# Autodesk Inventor assembly: carro_linear
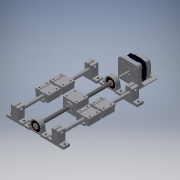
[picture p0: Inventor's stored thumbnail of the model, 180x180]
Saved by Autodesk Inventor 2018 (Build 220112000, 112)
## iProperties
Created: 2018-09-21
Part Number: carro_linear
Material: Genérico
Document SubType Name: Assembly
Designer: Georgines
Author: Georgines
## Documents named in this file (10)
- C:\Users\Georgines\Documents\EstacaoBGA\Peças 3D\carro_linear.iam
- C:\Users\Georgines\Documents\EstacaoBGA\Peças 3D\CastanhaTR8.ipt
- C:\Users\Georgines\Documents\EstacaoBGA\Peças 3D\FusoTrapezoidal_8mmx200mm.ipt
- C:\Users\Georgines\Documents\EstacaoBGA\Peças 3D\kp08.ipt
- C:\Users\Georgines\Documents\EstacaoBGA\Peças 3D\NEMA-17_17HS4401.ipt
- C:\Users\Georgines\Documents\EstacaoBGA\Peças 3D\SCS8UU.iam
- C:\Users\Georgines\Documents\EstacaoBGA\Peças 3D\Sk8.ipt
- C:\Users\Georgines\Documents\EstacaoBGA\Peças 3D\SuporteCastanhaTr8.ipt
- C:\Users\Georgines\Documents\EstacaoBGA\Peças 3D\SuporteLMotorNema17.ipt
- C:\Users\Georgines\Documents\EstacaoBGA\Peças 3D\GuiaLinear_8mmx200mm.ipt
## Components (17 placed, 9 different names)
1. FusoTrapezoidal_8mmx200mm:1 — Coincidência:9, Coincidência:10, Alinhamento:10, Inserir:1
2. kp08:1 — Alinhamento:7, Coincidência:9, Alinhamento:9, Alinhamento:10, Alinhamento:20, Alinhamento:23, Coincidência:13, Coincidência:14
3. kp08:2 — Alinhamento:8, Coincidência:10, Alinhamento:11, Alinhamento:16, Alinhamento:21, Alinhamento:22
4. NEMA-17_17HS4401:1 — Coincidência:11, Coincidência:12
5. GuiaLinear_8mmx200mm:1 — Coincidência:2, Alinhamento:2, Coincidência:4, Alinhamento:4, Coincidência:5, Coincidência:8
6. GuiaLinear_8mmx200mm:2 — Coincidência:1, Alinhamento:1, Coincidência:3, Alinhamento:3, Coincidência:6, Coincidência:7
7. Sk8:1 — Coincidência:1, Alinhamento:1, Alinhamento:7, Alinhamento:9, Alinhamento:23, Coincidência:14
8. Sk8:2 — Coincidência:2, Alinhamento:2, Alinhamento:20, Coincidência:13
9. Sk8:3 — Coincidência:3, Alinhamento:3, Alinhamento:5, Alinhamento:6, Alinhamento:8, Alinhamento:11, Alinhamento:22
10. Sk8:4 — Coincidência:4, Alinhamento:4, Alinhamento:5, Alinhamento:6, Alinhamento:21
11. SCS8UU:1 [sub-assembly] — Coincidência:8, Alinhamento:12, Alinhamento:13, Alinhamento:17, Alinhamento:24
12. SCS8UU:2 [sub-assembly] — Coincidência:7, Alinhamento:14, Alinhamento:15, Alinhamento:17, Alinhamento:24, Coincidência:15
13. SCS8UU:3 [sub-assembly] — Coincidência:5, Alinhamento:12, Alinhamento:13, Alinhamento:18, Alinhamento:19, Alinhamento:25
14. SCS8UU:4 [sub-assembly] — Coincidência:6, Alinhamento:14, Alinhamento:15, Alinhamento:18, Alinhamento:19, Coincidência:15
15. SuporteLMotorNema17:1 — Coincidência:11, Coincidência:12, Alinhamento:16
16. SuporteCastanhaTr8:1 — Coincidência:16, Coincidência:17, Alinhamento:25
17. CastanhaTR8:1 — Inserir:1, Coincidência:16, Coincidência:17
## Relationships (43: Flush 25, Mate 17, Insert 1)
- Coincidência:1 [Mate]: GuiaLinear_8mmx200mm:2 ↔ Sk8:1
- Coincidência:2 [Mate]: GuiaLinear_8mmx200mm:1 ↔ Sk8:2
- Alinhamento:1 [Flush]: GuiaLinear_8mmx200mm:2 ↔ Sk8:1
- Alinhamento:2 [Flush]: GuiaLinear_8mmx200mm:1 ↔ Sk8:2
- Coincidência:3 [Mate]: GuiaLinear_8mmx200mm:2 ↔ Sk8:3
- Coincidência:4 [Mate]: GuiaLinear_8mmx200mm:1 ↔ Sk8:4
- Alinhamento:3 [Flush]: GuiaLinear_8mmx200mm:2 ↔ Sk8:3
- Alinhamento:4 [Flush]: GuiaLinear_8mmx200mm:1 ↔ Sk8:4
- Alinhamento:5 [Flush]: Sk8:3 ↔ Sk8:4
- Alinhamento:6 [Flush]: Sk8:3 ↔ Sk8:4
- Coincidência:5 [Mate]: GuiaLinear_8mmx200mm:1 ↔ SCS8UU:3
- Coincidência:6 [Mate]: GuiaLinear_8mmx200mm:2 ↔ SCS8UU:4
- Coincidência:7 [Mate]: GuiaLinear_8mmx200mm:2 ↔ SCS8UU:2
- Coincidência:8 [Mate]: GuiaLinear_8mmx200mm:1 ↔ SCS8UU:1
- Alinhamento:7 [Flush]: kp08:1 ↔ Sk8:1
- Alinhamento:8 [Flush]: kp08:2 ↔ Sk8:3
- Coincidência:9 [Mate]: FusoTrapezoidal_8mmx200mm:1 ↔ kp08:1
- Coincidência:10 [Mate]: FusoTrapezoidal_8mmx200mm:1 ↔ kp08:2
- Alinhamento:9 [Flush]: kp08:1 ↔ Sk8:1
- Alinhamento:10 [Flush]: FusoTrapezoidal_8mmx200mm:1 ↔ kp08:1
- Alinhamento:11 [Flush]: kp08:2 ↔ Sk8:3
- Alinhamento:12 [Flush]: SCS8UU:1 ↔ SCS8UU:3
- Alinhamento:13 [Flush]: SCS8UU:1 ↔ SCS8UU:3
- Alinhamento:14 [Flush]: SCS8UU:2 ↔ SCS8UU:4
- Alinhamento:15 [Flush]: SCS8UU:2 ↔ SCS8UU:4
- Coincidência:11 [Mate]: NEMA-17_17HS4401:1 ↔ SuporteLMotorNema17:1
- Coincidência:12 [Mate]: NEMA-17_17HS4401:1 ↔ SuporteLMotorNema17:1
- Alinhamento:16 [Flush]: kp08:2 ↔ SuporteLMotorNema17:1
- Alinhamento:17 [Flush]: SCS8UU:1 ↔ SCS8UU:2
- Alinhamento:18 [Flush]: SCS8UU:3 ↔ SCS8UU:4
- Alinhamento:19 [Flush]: SCS8UU:3 ↔ SCS8UU:4
- Alinhamento:20 [Flush]: kp08:1 ↔ Sk8:2
- Alinhamento:21 [Flush]: kp08:2 ↔ Sk8:4
- Alinhamento:22 [Flush]: kp08:2 ↔ Sk8:3
- Alinhamento:23 [Flush]: kp08:1 ↔ Sk8:1
- Coincidência:13 [Mate] (2 mm): kp08:1 ↔ Sk8:2
- Coincidência:14 [Mate] (2 mm): kp08:1 ↔ Sk8:1
- Inserir:1: FusoTrapezoidal_8mmx200mm:1 ↔ CastanhaTR8:1
- Alinhamento:24 [Flush]: SCS8UU:1 ↔ SCS8UU:2
- Coincidência:15 [Mate] (5 mm): SCS8UU:2 ↔ SCS8UU:4
- Coincidência:16 [Mate]: SuporteCastanhaTr8:1 ↔ CastanhaTR8:1
- Coincidência:17 [Mate]: SuporteCastanhaTr8:1 ↔ CastanhaTR8:1
- Alinhamento:25 [Flush]: SCS8UU:3 ↔ SuporteCastanhaTr8:1
